# Autodesk Inventor assembly: Computer Box Assembly Rev2
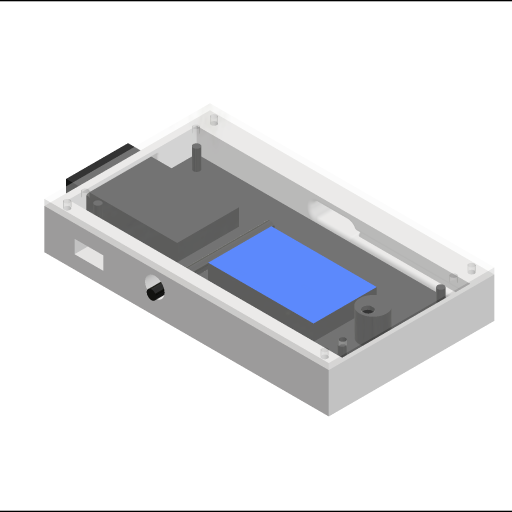
[picture p0: Inventor's stored thumbnail of the model, 512x512]
Saved by Autodesk Inventor 2023 (Build 270158000, 158)
## iProperties
Created: 2023-01-21
Part Number: Computer Box Assembly Rev2
Document SubType Name: Assembly
Designer: kamer
Author: kamer
## Documents named in this file (4)
- X:\Storage\Documents\ME 306 Heat Transfer Project Files\CAD\Computer Box Assembly Rev2.iam
- X:\Storage\Documents\ME 306 Heat Transfer Project Files\CAD\Computer Box Base Rev2.ipt
- X:\Storage\Documents\ME 306 Heat Transfer Project Files\CAD\Circuit Board Mockup.ipt
- X:\Storage\Documents\ME 306 Heat Transfer Project Files\CAD\2023 1 17 Computer Box Door.ipt
## Components (3 placed, 3 different names)
1. Computer Box Base Rev2:1 — Mate:1, Mate:2, Mate:3, Mate:4, Mate:5, Mate:6
2. Circuit Board Mockup:1 — Mate:1, Mate:2, Mate:3
3. 2023 1 17 Computer Box Door:1 — Mate:4, Mate:5, Mate:6
## Relationships (6: Mate 6)
- Mate:1: Computer Box Base Rev2:1 ↔ Circuit Board Mockup:1
- Mate:2: Computer Box Base Rev2:1 ↔ Circuit Board Mockup:1
- Mate:3: Computer Box Base Rev2:1 ↔ Circuit Board Mockup:1
- Mate:4: Computer Box Base Rev2:1 ↔ 2023 1 17 Computer Box Door:1
- Mate:5: Computer Box Base Rev2:1 ↔ 2023 1 17 Computer Box Door:1
- Mate:6: Computer Box Base Rev2:1 ↔ 2023 1 17 Computer Box Door:1
